# Autodesk Inventor assembly: Корпус ноги в сборе_MIR
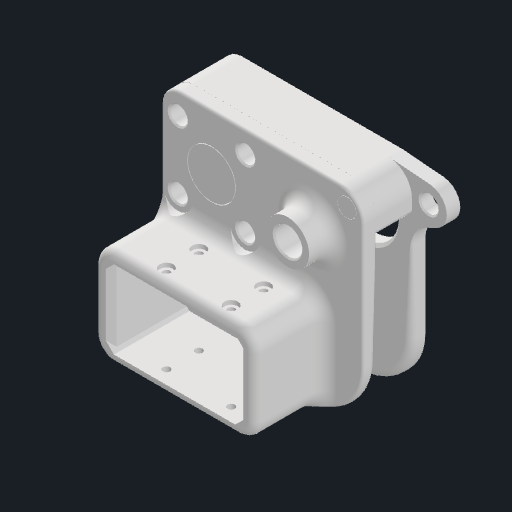
[picture p0: Inventor's stored thumbnail of the model, 512x512]
Saved by Autodesk Inventor 2025 (Build 290162010, 162A)
## iProperties
Created: 2025-01-17
Part Number: Корпус ноги в сборе_MIR
Document SubType Name: Assembly
Designer: Edward_Higgins
Author: Edward_Higgins
## Documents named in this file (3)
- D:\Users\Edward_Higgins\Desktop\ZAVOD\Робот Сколково\Корпус ноги в сборе_MIR.iam
- D:\Users\Edward_Higgins\Desktop\ZAVOD\Робот Сколково\Корпус ноги 2_MIR.ipt
- D:\Users\Edward_Higgins\Desktop\ZAVOD\Робот Сколково\Пластина корпуса ноги_MIR.ipt
## Components (2 placed, 2 different names)
1. Корпус ноги 2_MIR:1 — Совмещение:2, Совмещение:1, Совмещение:5, Совмещение:4, Совмещение:3
2. Пластина корпуса ноги_MIR:1 — Совмещение:5, Совмещение:4, Совмещение:3
## Relationships (5: Mate 5)
- Совмещение:2 [Mate]: Корпус ноги 2_MIR:1
- Совмещение:1 [Mate]: Корпус ноги 2_MIR:1
- Совмещение:5 [Mate]: Корпус ноги 2_MIR:1 ↔ Пластина корпуса ноги_MIR:1
- Совмещение:4 [Mate]: Корпус ноги 2_MIR:1 ↔ Пластина корпуса ноги_MIR:1
- Совмещение:3 [Mate]: Корпус ноги 2_MIR:1 ↔ Пластина корпуса ноги_MIR:1
